# Autodesk Inventor assembly: Turret Shooter Assembly
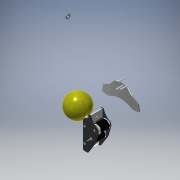
[picture p0: Inventor's stored thumbnail of the model, 180x180]
Saved by Autodesk Inventor 2019.4 (Build 234330000, 330)
## iProperties
Created: 2020-01-06
Part Number: Turret Shooter Assembly
Document SubType Name: Assembly
Designer: admin
Mass: 4067.01 g
Surface Area: 6466.54 cm^2
Volume: 4994.12 cm^3
Density: 0.814359 g/cm^3
Author: admin
## Documents named in this file (12)
- C:\Users\admin\Desktop\FRC 2020 Engineering\GitHub\7738-2020\Turret\Turret Shooter Assembly.iam
- C:\Users\admin\Desktop\FRC 2020 Engineering\GitHub\7738-2020\Turret\Omni Wheel\3_25_Omni-Directional_Wheel_217-4775.iam
- C:\Users\admin\Desktop\FRC 2020 Engineering\GitHub\7738-2020\Power Cell.ipt
- C:\Users\admin\Desktop\FRC 2020 Engineering\GitHub\7738-2020\Turret\Flywheel.ipt
- C:\Users\admin\Desktop\FRC 2020 Engineering\GitHub\7738-2020\Turret\Mini CIM\Mini_CIM_Motor_217-3371.ipt
- C:\Users\admin\Desktop\FRC 2020 Engineering\GitHub\7738-2020\CAD\Gearbox\F6800.ipt
- C:\Users\admin\Desktop\FRC 2020 Engineering\GitHub\7738-2020\Turret\Flywheel Bracket 1.ipt
- C:\Users\admin\Desktop\FRC 2020 Engineering\GitHub\7738-2020\Turret\Pivot Plate.ipt
- C:\Users\admin\Desktop\FRC 2020 Engineering\GitHub\7738-2020\Turret\Slewing Bearing.ipt
- C:\Users\admin\Desktop\FRC 2020 Engineering\GitHub\7738-2020\CAD\Gearbox\F6804.ipt
- C:\Users\admin\Desktop\FRC 2020 Engineering\GitHub\7738-2020\Turret\Ball Stop.ipt
- C:\Users\admin\Desktop\FRC 2020 Engineering\GitHub\7738-2020\Turret\Stopper Spacers.ipt
## Components (18 placed, 11 different names)
1. 3_25_Omni-Directional_Wheel_217-4775:1 [sub-assembly] — Mate:5, Mate:6
2. Power Cell:1 — Mate:14, Mate:15, Mate:16
3. Flywheel:1 — Mate:1, Mate:2, Mate:17, Mate:19
4. F6800:2 — Mate:2, Mate:4, Mate:9
5. Flywheel Bracket 1:1 — Mate:3, Mate:4, Mate:7, Mate:8, Mate:9, Mate:13, Angle:1, Mate:28, Flush:1
6. F6800:3 — Mate:1, Mate:27
7. F6800:5 — Mate:6, Mate:7, Mate:8
8. Pivot Plate:1 — Mate:31, Mate:32, Mate:33
9. Slewing Bearing:1
10. F6804:2
11. Ball Stop:1
12. Stopper Spacers:4
13. Stopper Spacers:5
14. Stopper Spacers:6
15. Mini_CIM_Motor_217-3371:4 — Mate:3, Mate:13, Mate:22, Mate:26
16. Mini_CIM_Motor_217-3371:5 — Mate:22, Mate:23, Mate:24, Mate:25
17. Flywheel Bracket 1:2 — Mate:24, Mate:25, Mate:26, Mate:27, Mate:28, Mate:29, Mate:30, Mate:31, Mate:32, Mate:33
18. F6800:6 — Mate:29, Mate:30
## Relationships (31: Mate 29, Angle 1, Flush 1)
- Mate:1: Flywheel:1 ↔ F6800:3
- Mate:2: Flywheel:1 ↔ F6800:2
- Mate:3: Flywheel Bracket 1:1 ↔ Mini_CIM_Motor_217-3371:4
- Mate:4: F6800:2 ↔ Flywheel Bracket 1:1
- Mate:5: 3_25_Omni-Directional_Wheel_217-4775:1
- Mate:6: 3_25_Omni-Directional_Wheel_217-4775:1 ↔ F6800:5
- Mate:7: Flywheel Bracket 1:1 ↔ F6800:5
- Mate:8 (0.2 mm): Flywheel Bracket 1:1 ↔ F6800:5
- Mate:9 (0.2 mm): F6800:2 ↔ Flywheel Bracket 1:1
- Mate:13: Flywheel Bracket 1:1 ↔ Mini_CIM_Motor_217-3371:4
- Mate:14: Power Cell:1
- Mate:15: Power Cell:1
- Mate:16: Power Cell:1
- Mate:17 (104.775 mm): Flywheel:1
- Mate:18 (104.775 mm)
- Angle:1 (0 deg): Flywheel Bracket 1:1
- Mate:19 (-25 mm): Flywheel:1
- Mate:20 (-65 mm)
- Mate:22 (72.5 mm): Mini_CIM_Motor_217-3371:4 ↔ Mini_CIM_Motor_217-3371:5
- Mate:23 (77.5 mm): Mini_CIM_Motor_217-3371:5
- Mate:24: Mini_CIM_Motor_217-3371:5 ↔ Flywheel Bracket 1:2
- Mate:25: Mini_CIM_Motor_217-3371:5 ↔ Flywheel Bracket 1:2
- Mate:26: Mini_CIM_Motor_217-3371:4 ↔ Flywheel Bracket 1:2
- Mate:27 (0.2 mm): F6800:3 ↔ Flywheel Bracket 1:2
- Mate:28 (95 mm): Flywheel Bracket 1:1 ↔ Flywheel Bracket 1:2
- Flush:1 (47.5 mm): Flywheel Bracket 1:1
- Mate:29: Flywheel Bracket 1:2 ↔ F6800:6
- Mate:30 (0.2 mm): Flywheel Bracket 1:2 ↔ F6800:6
- Mate:31: Pivot Plate:1 ↔ Flywheel Bracket 1:2
- Mate:32: Pivot Plate:1 ↔ Flywheel Bracket 1:2
- Mate:33: Pivot Plate:1 ↔ Flywheel Bracket 1:2
